# Autodesk Inventor assembly: !gearbox
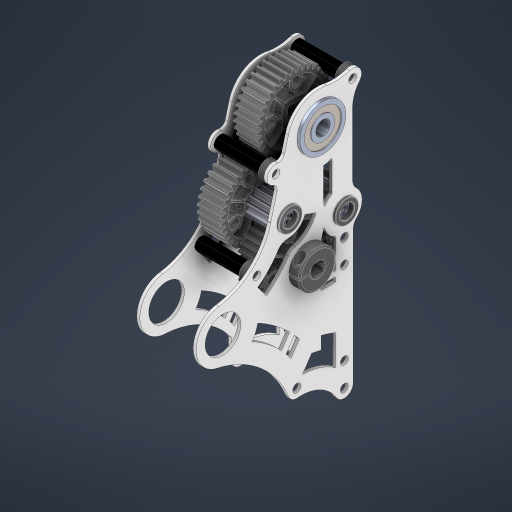
[picture p0: Inventor's stored thumbnail of the model, 512x512]
Saved by Autodesk Inventor 2024 (Build 280153000, 153)
## iProperties
Created: 2023-11-21
Part Number: !gearbox
Document SubType Name: Assembly
Designer: avere
Author: avere
## Documents named in this file (14)
- C:\Users\avere\Documents\rbp_cad\zoomba_v0.1\arm\!gearbox.iam
- C:\Users\avere\Documents\rbp_cad\zoomba_v0.1\chassis\custom_parts\reservoir_mount.ipt
- C:\Users\avere\Documents\rbp_cad\VEX-CAD-Inventor-1.41\Motion\Shaft HS\HS Bushing 0.1250.ipt
- C:\Users\avere\Documents\rbp_cad\VEX-CAD-Inventor-1.41\Motion\Gears\HS Gear\HS 12T Gear, No Insert.iam
- C:\Users\avere\Documents\rbp_cad\VEX-CAD-Inventor-1.41\Motion\Gears\HS Gear.iam
- C:\Users\avere\Documents\rbp_cad\VEX-CAD-Inventor-1.41\Motion\Gears\HS Gear\HS 36T Gear, No Insert.iam
- C:\Users\avere\Documents\rbp_cad\VEX-CAD-Inventor-1.41\Motion\Reference Files\Ball Bearing.ipt
- C:\Users\avere\Documents\rbp_cad\VEX-CAD-Inventor-1.41\Structure\Standoff\Standoff 1.00.ipt
- C:\Users\avere\Documents\rbp_cad\VEX-CAD-Inventor-1.41\Structure\Standoff.ipt
- C:\Users\avere\Documents\rbp_cad\VEX-CAD-Inventor-1.41\Motion\Spacers\Spacer Nylon .375 OD\NSpacer .375 OD x .125.ipt
- C:\Users\avere\Documents\rbp_cad\VEX-CAD-Inventor-1.41\Motion\Spacers\Spacer Nylon .375 OD.ipt
- C:\Users\avere\Documents\rbp_cad\VEX-CAD-Inventor-1.41\Motion\Shaft HS\Low Profile HS Shaft Collar.ipt
- C:\Users\avere\Documents\rbp_cad\VEX-CAD-Inventor-1.41\Motion\Shaft HS\HS Shaft Collar.ipt
- C:\Users\avere\Documents\rbp_cad\zoomba_v0.1\chassis\custom_parts\reservoir_mount_inner.ipt
## Components (21 placed, 10 different names)
1. reservoir_mount:1 — Insert:19, Mate:1
2. HS Bushing 0.1250:1
3. HS Bushing 0.1250:2
4. HS Bushing 0.1250:3
5. HS 12T Gear, No Insert:1 [sub-assembly]
6. HS 12T Gear, No Insert:2 [sub-assembly]
7. HS 36T Gear, No Insert:3 [sub-assembly]
8. HS 36T Gear, No Insert:4 [sub-assembly]
9. HS 12T Gear, No Insert:5 [sub-assembly]
10. Ball Bearing:1
11. Standoff 1.00:1
12. NSpacer .375 OD x .125:1
13. Standoff 1.00:2
14. NSpacer .375 OD x .125:2
15. Standoff 1.00:3
16. NSpacer .375 OD x .125:3
17. HS 36T Gear, No Insert:6 [sub-assembly] — Insert:21
18. Low Profile HS Shaft Collar:1
19. HS Shaft Collar:1
20. reservoir_mount_inner:1 — Insert:19, Mate:1, Insert:20
21. Ball Bearing:2 — Insert:20, Insert:21
## Relationships (20: Insert 19, Mate 1)
- [Insert]: reservoir_mount:1 ↔ HS Bushing 0.1250:2
- [Insert]: reservoir_mount:1 ↔ HS Bushing 0.1250:3
- [Insert]: reservoir_mount:1 ↔ HS Bushing 0.1250:1
- [Insert] (1.5875 mm): HS Bushing 0.1250:1 ↔ HS 12T Gear, No Insert:1
- [Insert] (1.5875 mm): HS Bushing 0.1250:2 ↔ HS 36T Gear, No Insert:3
- [Insert]: HS 12T Gear, No Insert:2 ↔ HS 36T Gear, No Insert:3
- [Insert] (14.2875 mm): HS Bushing 0.1250:3 ↔ HS 36T Gear, No Insert:4
- [Insert]: HS 36T Gear, No Insert:4 ↔ HS 12T Gear, No Insert:5
- [Insert]: Standoff 1.00:1 ↔ NSpacer .375 OD x .125:1
- [Insert]: reservoir_mount:1 ↔ NSpacer .375 OD x .125:1
- [Insert]: Standoff 1.00:2 ↔ NSpacer .375 OD x .125:2
- [Insert]: reservoir_mount:1 ↔ NSpacer .375 OD x .125:2
- [Insert]: Standoff 1.00:3 ↔ NSpacer .375 OD x .125:3
- [Insert]: reservoir_mount:1 ↔ NSpacer .375 OD x .125:3
- [Insert]: reservoir_mount:1 ↔ Ball Bearing:1
- [Insert]: HS Bushing 0.1250:2 ↔ Low Profile HS Shaft Collar:1
- Insert:19 (28.575 mm): reservoir_mount:1 ↔ reservoir_mount_inner:1
- Mate:1: reservoir_mount:1 ↔ reservoir_mount_inner:1
- Insert:20: reservoir_mount_inner:1 ↔ Ball Bearing:2
- Insert:21: HS 36T Gear, No Insert:6 ↔ Ball Bearing:2
## Named parameters: d416_d414 = 0 mm, d418_d414 = 0 mm
